# Autodesk Inventor assembly: драйвер
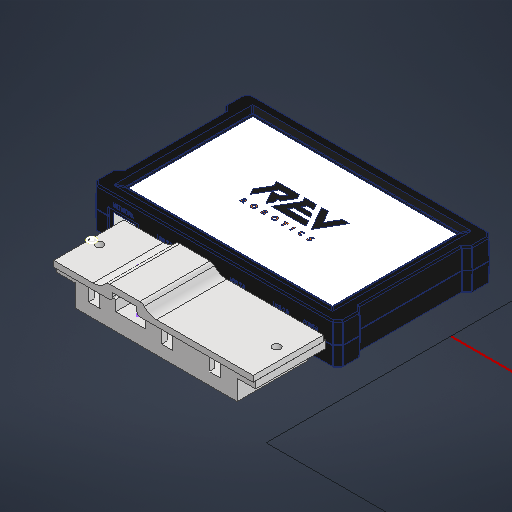
[picture p0: Inventor's stored thumbnail of the model, 512x512]
Saved by Autodesk Inventor 2026.2 (Build 302298000, 298)
## iProperties
Created: 2025-03-13
Part Number: драйвер
Document SubType Name: Assembly
Designer: Phantom
Author: Phantom
## Documents named in this file (6)
- C:\Users\Phantom\Desktop\Phantom16950\драйвер.iam
- C:\Users\Phantom\Desktop\Phantom16950\REV-31-1596.ipt
- C:\Users\Phantom\Desktop\Phantom16950\драйвер.ipt
- C:\Users\Phantom\Desktop\Phantom16950\драйвер 2.ipt
- C:\Users\Phantom\Desktop\Phantom16950\16950 2часть\16950 1.3часть\16950 1.3часть.ipt
- C:\Users\Phantom\Desktop\Phantom16950\16950 2часть\16950 2.3часть\16950 2.3часть.ipt
## Components (5 placed, 5 different names)
1. REV-31-1596:1 — Совмещение:2, Совмещение:3, Совмещение:6, Совмещение:9, Заподлицо:9
2. драйвер:1 — Совмещение:2, Совмещение:3, Совмещение:4, Совмещение:5, Заподлицо:7
3. драйвер 2:1 — Совмещение:4, Совмещение:5, Заподлицо:7
4. 16950 1.3часть:1 — Совмещение:7, Совмещение:8, Заподлицо:8
5. 16950 2.3часть:1 — Совмещение:6, Совмещение:7, Совмещение:8, Совмещение:9, Заподлицо:8, Заподлицо:9
## Relationships (11: Mate 8, Flush 3)
- Совмещение:2 [Mate]: REV-31-1596:1 ↔ драйвер:1
- Совмещение:3 [Mate]: REV-31-1596:1 ↔ драйвер:1
- Совмещение:4 [Mate]: драйвер:1 ↔ драйвер 2:1
- Совмещение:5 [Mate]: драйвер:1 ↔ драйвер 2:1
- Заподлицо:7 [Flush]: драйвер:1 ↔ драйвер 2:1
- Совмещение:6 [Mate]: REV-31-1596:1 ↔ 16950 2.3часть:1
- Совмещение:7 [Mate]: 16950 1.3часть:1 ↔ 16950 2.3часть:1
- Совмещение:8 [Mate]: 16950 1.3часть:1 ↔ 16950 2.3часть:1
- Совмещение:9 [Mate]: REV-31-1596:1 ↔ 16950 2.3часть:1
- Заподлицо:8 [Flush]: 16950 1.3часть:1 ↔ 16950 2.3часть:1
- Заподлицо:9 [Flush]: REV-31-1596:1 ↔ 16950 2.3часть:1
